# Autodesk Inventor assembly: XEnd
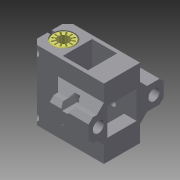
[picture p0: Inventor's stored thumbnail of the model, 180x180]
Saved by Autodesk Inventor 2015 (Build 190159000, 159)
## iProperties
Created: 2014-08-10
Part Number: XEnd
Document SubType Name: Assembly
Designer: Jack
Author: Jack
## Documents named in this file (3)
- C:\Users\Jack\ownCloud\Projects\CoreXY\InventorModel\XAxis\XEnd.iam
- C:\Users\Jack\ownCloud\Projects\CoreXY\InventorModel\XAxis\XEnd.ipt
- C:\Users\Jack\ownCloud\Projects\CoreXY\InventorModel\Hardware\Bearings \Igus\BushingIgusRJM-01-08.ipt
## Components (3 placed, 2 different names)
1. XEnd:1 — Mate:2, Mate:3, Mate:4, Mate:5
2. BushingIgusRJM-01-08:2 — Mate:2, Mate:4
3. BushingIgusRJM-01-08:3 — Mate:3, Mate:5
## Relationships (4: Mate 4)
- Mate:2: XEnd:1 ↔ BushingIgusRJM-01-08:2
- Mate:3: XEnd:1 ↔ BushingIgusRJM-01-08:3
- Mate:4: XEnd:1 ↔ BushingIgusRJM-01-08:2
- Mate:5: XEnd:1 ↔ BushingIgusRJM-01-08:3
